# Autodesk Inventor assembly: Fingertip assembly final
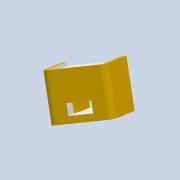
[picture p0: Inventor's stored thumbnail of the model, 180x180]
Saved by Autodesk Inventor 2020 (Build 240168000, 168)
## iProperties
Created: 2020-02-13
Part Number: Fingertip assembly final
Document SubType Name: Assembly
Designer: kaipa
Author: kaipa
## Documents named in this file (4)
- C:\Users\sami_\Documents\V1.5\Workgroups\NotInProject\RING\Fingertip assembly final.iam
- C:\Users\sami_\Documents\V1.5\Workgroups\NotInProject\RING\L3.ipt
- C:\Users\sami_\Documents\V1.5\Workgroups\NotInProject\RING\fingertip lid 5.ipt
- C:\Users\sami_\Documents\V1.5\Workgroups\NotInProject\1D Fingertip skeleton.ipt
## Components (4 placed, 3 different names)
1. fingertip lid 5:1
2. 1D Fingertip skeleton:1 — Rigid:3
3. fingertip lid 5:2
4. L3:1 — Rigid:3
## Relationships (3: WeldJoint 3)
- [WeldJoint]: fingertip lid 5:1 ↔ 1D Fingertip skeleton:1
- [WeldJoint]: 1D Fingertip skeleton:1 ↔ fingertip lid 5:2
- Rigid:3 [WeldJoint]: 1D Fingertip skeleton:1 ↔ L3:1
